# Autodesk Inventor assembly: Robot Chassis - Short and Narrow
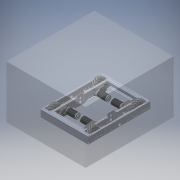
[picture p0: Inventor's stored thumbnail of the model, 180x180]
Saved by Autodesk Inventor 2017 (Build 210142000, 142)
## iProperties
Created: 2017-01-10
Part Number: Robot Chassis - Short and Narrow
Document SubType Name: Assembly
Designer: Roksbot
Author: Roksbot
## Documents named in this file (5)
- C:\Users\Roksbot\Documents\Inventor\2017 Robot\Robot Chassis - Short and Narrow.iam
- C:\Users\Roksbot\Documents\Inventor\2017 Robot\Short Build Volume.ipt
- C:\Users\Roksbot\Documents\Inventor\2017 Robot\Tall Build Volume.ipt
- C:\Users\Roksbot\Documents\Inventor\2017 Robot\Robot Chassis Half.iam
- C:\Users\Roksbot\Documents\Inventor\2017 Robot\End Sheet - 21.5.ipt
## Components (6 placed, 4 different names)
1. Short Build Volume:1 — Flush:5, Flush:6, Flush:7, Flush:8, Flush:9
2. Tall Build Volume:1 — Flush:5, Flush:6, Flush:7, Flush:12
3. Robot Chassis Half:1 [sub-assembly] — Flush:8, Flush:9, Flush:10, Flush:11, Mate:1, Flush:12, Insert:1, Insert:3
4. Robot Chassis Half:2 [sub-assembly] — Flush:10, Flush:11, Mate:1, Insert:2, Insert:4
5. End Sheet - 21.5:1 — Insert:2, Insert:3
6. End Sheet - 21.5:2 — Insert:1, Insert:4
## Relationships (13: Flush 8, Insert 4, Mate 1)
- Flush:5: Short Build Volume:1 ↔ Tall Build Volume:1
- Flush:6: Short Build Volume:1 ↔ Tall Build Volume:1
- Flush:7: Short Build Volume:1 ↔ Tall Build Volume:1
- Flush:8 (88.9 mm): Short Build Volume:1 ↔ Robot Chassis Half:1
- Flush:9 (-38.1 mm): Short Build Volume:1 ↔ Robot Chassis Half:1
- Flush:10: Robot Chassis Half:1 ↔ Robot Chassis Half:2
- Flush:11: Robot Chassis Half:1 ↔ Robot Chassis Half:2
- Mate:1 (533.4 mm): Robot Chassis Half:1 ↔ Robot Chassis Half:2
- Flush:12 (177.8 mm): Tall Build Volume:1 ↔ Robot Chassis Half:1
- Insert:1: Robot Chassis Half:1 ↔ End Sheet - 21.5:2
- Insert:2: Robot Chassis Half:2 ↔ End Sheet - 21.5:1
- Insert:3: Robot Chassis Half:1 ↔ End Sheet - 21.5:1
- Insert:4: Robot Chassis Half:2 ↔ End Sheet - 21.5:2
